# Autodesk Inventor assembly: Head
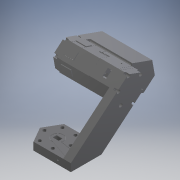
[picture p0: Inventor's stored thumbnail of the model, 180x180]
Saved by Autodesk Inventor 2017 (Build 210142000, 142)
## iProperties
Created: 2018-10-18
Part Number: Head
Document SubType Name: Assembly
Designer: Dell
Author: Dell
## Documents named in this file (6)
- C:\Users\Dell\Documents\GitHub\tr2\Head\Head.iam
- C:\Users\Dell\Documents\GitHub\tr2\Head\Orbbec Astra\Orbbec Astra.iam
- C:\Users\Dell\Documents\GitHub\tr2\Head\HA07.ipt
- C:\Users\Dell\Documents\GitHub\tr2\Head\HA08.ipt
- C:\Users\Dell\Documents\GitHub\tr2\Actuator 1.3\Actuator 1.3.iam
- C:\Users\Dell\Documents\GitHub\tr2\Head\HA09.ipt
## Components (5 placed, 5 different names)
1. Orbbec Astra:1 [sub-assembly] — Mate:58, Mate:59, Angle:1
2. HA07:1 — Mate:47, Mate:50, Mate:54, Mate:60, Mate:61, Mate:62, Mate:65, Mate:66, Angle:2, Mate:67
3. HA08:1 — Mate:58, Mate:59, Angle:1, Mate:63, Mate:64
4. Actuator 1.3:1 [sub-assembly] — Mate:60, Mate:61, Mate:62, Mate:63, Mate:64
5. HA09:1 — Mate:65, Mate:66, Angle:2, Mate:67
## Relationships (15: Mate 13, Angle 2)
- Mate:47: HA07:1
- Mate:50: HA07:1
- Mate:54: HA07:1
- Mate:58: Orbbec Astra:1 ↔ HA08:1
- Mate:59: Orbbec Astra:1 ↔ HA08:1
- Angle:1 (180 deg): Orbbec Astra:1 ↔ HA08:1
- Mate:60: HA07:1 ↔ Actuator 1.3:1
- Mate:61: HA07:1 ↔ Actuator 1.3:1
- Mate:62: HA07:1 ↔ Actuator 1.3:1
- Mate:63: HA08:1 ↔ Actuator 1.3:1
- Mate:64: HA08:1 ↔ Actuator 1.3:1
- Mate:65: HA07:1 ↔ HA09:1
- Mate:66: HA07:1 ↔ HA09:1
- Angle:2 (180 deg): HA07:1 ↔ HA09:1
- Mate:67: HA07:1 ↔ HA09:1
